# Autodesk Inventor assembly: A_hips_001
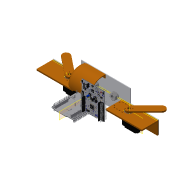
[picture p0: Inventor's stored thumbnail of the model, 180x180]
Saved by Autodesk Inventor 2016 (Build 200138000, 138)
## iProperties
Created: 2016-02-25
Part Number: A_hips_001
Document SubType Name: Assembly
Designer: Mateusz
Author: Mateusz
## Documents named in this file (11)
- D:\PROJECTS\2016_biped\hermes\mechanics_tmp\A_hips_001.iam
- D:\PROJECTS\2016_biped\hermes\mechanics_tmp\P_hips_001.ipt
- D:\PROJECTS\2016_biped\hermes\mechanics_tmp\P_hips02_001.ipt
- D:\PROJECTS\2016_biped\hermes\mechanics_tmp\AX-12A.iam
- D:\PROJECTS\2016_biped\hermes\mechanics_tmp\P_arm01_001.ipt
- D:\PROJECTS\2016_biped\hermes\mechanics_tmp\nucleo_boardNUCLEO-F411RE.iam
- D:\PROJECTS\2016_biped\hermes\mechanics_tmp\nucleo_board_as_part_4.ipt
- C:\Users\Mateusz\Documents\Inventor\Content Center Files\R2016\en-US\DIN 934\DIN 934 - M10 x 1.5.ipt
- C:\Users\Mateusz\Documents\Inventor\Content Center Files\R2016\en-US\DIN 125-1  A\DIN 125 - A 10.5.ipt
- D:\PROJECTS\2016_biped\hermes\mechanics_tmp\P_hips02_001_MIR.ipt
- D:\PROJECTS\2016_biped\hermes\mechanics_tmp\P_hips03_001.ipt
## Components (14 placed, 10 different names)
1. P_hips_001:1 — Mate:1, Mate:2, Flush:1, Mate:5, Insert:3, Insert:4, Mate:21
2. P_hips02_001:1 — Mate:3, Mate:4, Mate:5, Mate:6, Angle:1, Mate:7, Mate:8, Mate:22
3. AX-12A:1 [sub-assembly] — Mate:6, Angle:1, Mate:7, Mate:8, Mate:9, Mate:10, Mate:11
4. P_arm01_001:1 — Mate:9, Mate:10, Mate:11
5. nucleo_boardNUCLEO-F411RE:1 [sub-assembly]
6. nucleo_board_as_part_4:1 — Mate:12, Flush:2, Mate:22
7. DIN 934 - replaced by DIN EN 24032/28673/28674 M10:1 — Insert:1
8. DIN 125-1 A A 10.5:1 — Insert:1, Insert:3
9. DIN 934 - replaced by DIN EN 24032/28673/28674 M10:2
10. DIN 125-1 A A 10.5:2 — Insert:4
11. P_hips02_001_MIR:1 — Mate:14, Flush:3, Mate:15, Mate:16, Angle:2, Mate:17, Mate:21
12. AX-12A:2 [sub-assembly] — Mate:15, Mate:16, Angle:2, Mate:17, Mate:18, Mate:19, Mate:20
13. P_arm01_001:2 — Mate:18, Mate:19, Mate:20
14. P_hips03_001:1 — Flush:4
## Relationships (31: Mate 21, Flush 4, Insert 4, Angle 2)
- Mate:1: P_hips_001:1
- Mate:2: P_hips_001:1
- Flush:1: P_hips_001:1
- Mate:3: P_hips02_001:1
- Mate:4: P_hips02_001:1
- Mate:5: P_hips_001:1 ↔ P_hips02_001:1
- Mate:6: P_hips02_001:1 ↔ AX-12A:1
- Angle:1 (180 deg): P_hips02_001:1 ↔ AX-12A:1
- Mate:7: P_hips02_001:1 ↔ AX-12A:1
- Mate:8: P_hips02_001:1 ↔ AX-12A:1
- Mate:9: AX-12A:1 ↔ P_arm01_001:1
- Mate:10: AX-12A:1 ↔ P_arm01_001:1
- Mate:11: AX-12A:1 ↔ P_arm01_001:1
- Mate:12: nucleo_board_as_part_4:1
- Flush:2: nucleo_board_as_part_4:1
- Insert:1: DIN 934 - replaced by DIN EN 24032/28673/28674 M10:1 ↔ DIN 125-1 A A 10.5:1
- [Insert]: DIN 934 - replaced by DIN EN 24032/28673/28674 M10:2 ↔ DIN 125-1 A A 10.5:2
- Insert:3: P_hips_001:1 ↔ DIN 125-1 A A 10.5:1
- Insert:4: P_hips_001:1 ↔ DIN 125-1 A A 10.5:2
- Mate:14: P_hips02_001_MIR:1
- Flush:3: P_hips02_001_MIR:1
- Mate:15: P_hips02_001_MIR:1 ↔ AX-12A:2
- Mate:16: P_hips02_001_MIR:1 ↔ AX-12A:2
- Angle:2 (180 deg): P_hips02_001_MIR:1 ↔ AX-12A:2
- Mate:17: P_hips02_001_MIR:1 ↔ AX-12A:2
- Mate:18: AX-12A:2 ↔ P_arm01_001:2
- Mate:19: AX-12A:2 ↔ P_arm01_001:2
- Mate:20: AX-12A:2 ↔ P_arm01_001:2
- Mate:21: P_hips_001:1 ↔ P_hips02_001_MIR:1
- Flush:4: P_hips03_001:1
- Mate:22: P_hips02_001:1 ↔ nucleo_board_as_part_4:1
## Named parameters: d26_d25 = 0 mm
